# Autodesk Inventor assembly: main_board
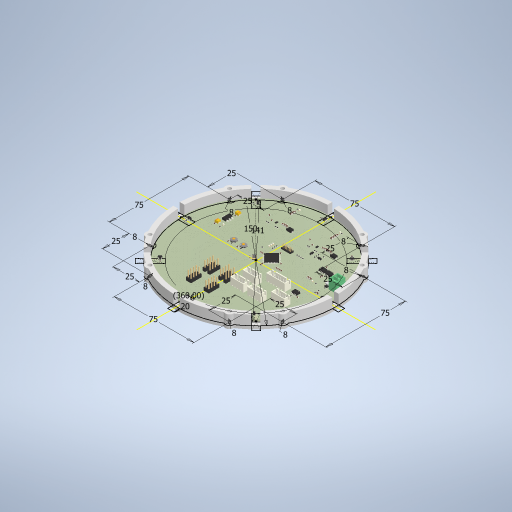
[picture p0: Inventor's stored thumbnail of the model, 512x512]
Saved by Autodesk Inventor 2024.3 (Build 283343000, 343)
## iProperties
Created: 2026-05-02
Part Number: main_board
Document SubType Name: Assembly
Designer: owozn
Author: owozn
## Documents named in this file (3)
- C:\Users\owozn\Documents\Nauka\Studia\mgr\Semestr_3\Magisterka\uMule\mechanics\subsets\attachments\main_board\main_board.iam
- C:\Users\owozn\Documents\Nauka\Studia\mgr\Semestr_3\Magisterka\uMule\mechanics\subsets\attachments\main_board\board_holder.ipt
- C:\Users\owozn\Documents\Nauka\Studia\mgr\Semestr_3\Magisterka\uMule\mechanics\subsets\attachments\main_board\uMule_board\uMule_board.iam
## Components (2 placed, 2 different names)
1. board_holder:1 — Mate:1, Mate:2
2. uMule_board:1 [sub-assembly] — Mate:1, Mate:2
## Relationships (2: Mate 2)
- Mate:1: board_holder:1 ↔ uMule_board:1
- Mate:2: board_holder:1 ↔ uMule_board:1
